# Autodesk Inventor assembly: outer
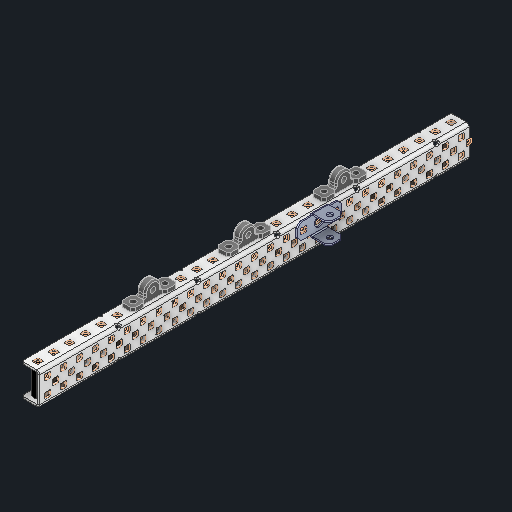
[picture p0: Inventor's stored thumbnail of the model, 512x512]
Saved by Autodesk Inventor 2024 (Build 280153000, 153)
## iProperties
Created: 2023-08-15
Part Number: outer
Document SubType Name: Assembly
Designer: avere
Author: avere
## Documents named in this file (11)
- D:\vex_robotics\hardware\cad\spades_v0.1\chassis\outer.iam
- D:\vex_robotics\hardware\cad\VEX-CAD-Inventor-1.41\Structure\C Channel\Aluminum 1x2x1\Alu C 1x2x1x27.ipt
- D:\vex_robotics\hardware\cad\VEX-CAD-Inventor-1.41\Motion\Shaft LS\Bearing Flat.ipt
- D:\vex_robotics\hardware\cad\VEX-CAD-Inventor-1.41\Motion\Spacers\Spacer Nylon .500 OD\NSpacer White .500 OD x .375.ipt
- D:\vex_robotics\hardware\cad\VEX-CAD-Inventor-1.41\Motion\Spacers\Spacer Nylon .500 OD\NSpacer White .500 OD x .500.ipt
- D:\vex_robotics\hardware\cad\VEX-CAD-Inventor-1.41\Motion\Shaft LS\LS Pillow Bearing Block.ipt
- D:\vex_robotics\hardware\cad\VEX-CAD-Inventor-1.41\Structure\Standoff\Standoff .875.ipt
- D:\vex_robotics\hardware\cad\VEX-CAD-Inventor-1.41\Structure\Standoff.ipt
- D:\vex_robotics\hardware\cad\VEX-CAD-Inventor-1.41\Motion\Spacers\Spacer Nylon .500 OD.ipt
- D:\vex_robotics\hardware\cad\VEX-CAD-Inventor-1.41\Motion\Shaft LS\Bearing Flat Low Profile.ipt
- D:\vex_robotics\hardware\cad\VEX-CAD-Inventor-1.41\Motion\Pneumatics\Cylinder Rod Pivot.ipt
## Components (15 placed, 8 different names)
1. Alu C 1x2x1x27:1 — Insert:7, Insert:8, Mate:7, Mate:8, Insert:10, Insert:16, Insert:17, Mate:12, Insert:18, Insert:19, Mate:13, Mate:14, Insert:20, Insert:21, Insert:22, Insert:23, Insert:24, Mate:15, Mate:16, Mate:17, Mate:18, Mate:19, Insert:25, Mate:20
2. Bearing Flat:1 — Insert:8, Mate:7
3. Bearing Flat:2 — Insert:7, Mate:8
4. NSpacer White .500 OD x .375:1 — Insert:10
5. NSpacer White .500 OD x .500:2
6. LS Pillow Bearing Block:1 — Insert:18, Mate:13
7. LS Pillow Bearing Block:2 — Insert:17, Mate:12
8. LS Pillow Bearing Block:3 — Insert:19, Mate:14
9. Standoff .875:1 — Insert:16
10. Bearing Flat Low Profile:1 — Insert:20, Mate:15
11. Bearing Flat Low Profile:2 — Insert:21, Mate:16
12. Bearing Flat Low Profile:3 — Insert:22, Mate:17
13. Bearing Flat Low Profile:4 — Insert:23, Mate:18
14. Bearing Flat Low Profile:5 — Insert:24, Mate:19
15. Cylinder Rod Pivot:1 — Insert:25, Mate:20
## Relationships (25: Insert 14, Mate 11)
- Insert:7: Alu C 1x2x1x27:1 ↔ Bearing Flat:2
- Insert:8: Alu C 1x2x1x27:1 ↔ Bearing Flat:1
- Mate:7: Alu C 1x2x1x27:1 ↔ Bearing Flat:1
- Mate:8: Alu C 1x2x1x27:1 ↔ Bearing Flat:2
- [Insert]: NSpacer White .500 OD x .375:1 ↔ NSpacer White .500 OD x .500:2
- Insert:10: Alu C 1x2x1x27:1 ↔ NSpacer White .500 OD x .375:1
- Insert:16: Alu C 1x2x1x27:1 ↔ Standoff .875:1
- Insert:17: Alu C 1x2x1x27:1 ↔ LS Pillow Bearing Block:2
- Mate:12: Alu C 1x2x1x27:1 ↔ LS Pillow Bearing Block:2
- Insert:18: Alu C 1x2x1x27:1 ↔ LS Pillow Bearing Block:1
- Insert:19: Alu C 1x2x1x27:1 ↔ LS Pillow Bearing Block:3
- Mate:13: Alu C 1x2x1x27:1 ↔ LS Pillow Bearing Block:1
- Mate:14: Alu C 1x2x1x27:1 ↔ LS Pillow Bearing Block:3
- Insert:20: Alu C 1x2x1x27:1 ↔ Bearing Flat Low Profile:1
- Insert:21: Alu C 1x2x1x27:1 ↔ Bearing Flat Low Profile:2
- Insert:22: Alu C 1x2x1x27:1 ↔ Bearing Flat Low Profile:3
- Insert:23: Alu C 1x2x1x27:1 ↔ Bearing Flat Low Profile:4
- Insert:24: Alu C 1x2x1x27:1 ↔ Bearing Flat Low Profile:5
- Mate:15: Alu C 1x2x1x27:1 ↔ Bearing Flat Low Profile:1
- Mate:16: Alu C 1x2x1x27:1 ↔ Bearing Flat Low Profile:2
- Mate:17: Alu C 1x2x1x27:1 ↔ Bearing Flat Low Profile:3
- Mate:18: Alu C 1x2x1x27:1 ↔ Bearing Flat Low Profile:4
- Mate:19: Alu C 1x2x1x27:1 ↔ Bearing Flat Low Profile:5
- Insert:25: Alu C 1x2x1x27:1 ↔ Cylinder Rod Pivot:1
- Mate:20: Alu C 1x2x1x27:1 ↔ Cylinder Rod Pivot:1
